# Autodesk Inventor assembly: H-Shaped-Assembly
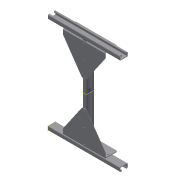
[picture p0: Inventor's stored thumbnail of the model, 180x180]
Saved by Autodesk Inventor 2015 (Build 190159000, 159)
## iProperties
Created: 2015-01-24
Part Number: H-Shaped-Assembly
Document SubType Name: Assembly
Designer: Peter
Author: Peter
## Documents named in this file (4)
- T:\FILES\FIRST-Team-1719-CAD-Team\2015 Robot CAD\Two Lifters and Lifter Super Structure\Lifter Super Structure\Tower\H-Shaped-Assembly\H-Shaped-Assembly.iam
- T:\FILES\FIRST-Team-1719-CAD-Team\2015 Robot CAD\Two Lifters and Lifter Super Structure\Lifter Super Structure\Tower\H-Shaped-Assembly\Horizontal-Center-Brace-H-Shape.ipt
- T:\FILES\FIRST-Team-1719-CAD-Team\2015 Robot CAD\Two Lifters and Lifter Super Structure\Lifter Super Structure\Tower\H-Shaped-Assembly\Horizontal-Unistrut-Tower-Connector-19-25.ipt
- T:\FILES\FIRST-Team-1719-CAD-Team\2015 Robot CAD\Two Lifters and Lifter Super Structure\Lifter Super Structure\Tower\H-Shaped-Assembly\Horizontal-Unistrut-Tower-Connector-15.ipt
## Components (5 placed, 3 different names)
1. Horizontal-Unistrut-Tower-Connector-19-25:1 — Mate:7, Mate:8, Mate:9
2. Horizontal-Unistrut-Tower-Connector-15:1 — Mate:1, Flush:1, Mate:2, Mate:5
3. Horizontal-Center-Brace-H-Shape:2 — Mate:1, Flush:1, Mate:2, Flush:3, Mate:6
4. Horizontal-Unistrut-Tower-Connector-15:3 — Mate:5, Mate:8
5. Horizontal-Center-Brace-H-Shape:3 — Flush:3, Mate:6, Mate:7, Mate:9
## Relationships (12: Mate 9, Flush 3)
- Mate:1: Horizontal-Unistrut-Tower-Connector-15:1 ↔ Horizontal-Center-Brace-H-Shape:2
- Flush:1: Horizontal-Unistrut-Tower-Connector-15:1 ↔ Horizontal-Center-Brace-H-Shape:2
- Mate:2: Horizontal-Unistrut-Tower-Connector-15:1 ↔ Horizontal-Center-Brace-H-Shape:2
- [Mate] (2.54 mm): Horizontal-Unistrut-Tower-Connector-15:3 ↔ Horizontal-Center-Brace-H-Shape:3
- [Flush]: Horizontal-Unistrut-Tower-Connector-15:3 ↔ Horizontal-Center-Brace-H-Shape:3
- [Mate]: Horizontal-Unistrut-Tower-Connector-15:3 ↔ Horizontal-Center-Brace-H-Shape:3
- Flush:3: Horizontal-Center-Brace-H-Shape:2 ↔ Horizontal-Center-Brace-H-Shape:3
- Mate:5 (488.95 mm): Horizontal-Unistrut-Tower-Connector-15:1 ↔ Horizontal-Unistrut-Tower-Connector-15:3
- Mate:6: Horizontal-Center-Brace-H-Shape:2 ↔ Horizontal-Center-Brace-H-Shape:3
- Mate:7: Horizontal-Unistrut-Tower-Connector-19-25:1 ↔ Horizontal-Center-Brace-H-Shape:3
- Mate:8: Horizontal-Unistrut-Tower-Connector-19-25:1 ↔ Horizontal-Unistrut-Tower-Connector-15:3
- Mate:9: Horizontal-Unistrut-Tower-Connector-19-25:1 ↔ Horizontal-Center-Brace-H-Shape:3
## Named parameters: d3_d0 = 2.54 mm, d4_d1 = 0 mm, d5_d2 = 0 mm
